# Autodesk Inventor assembly: HorquillaSuperior
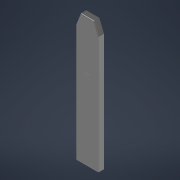
[picture p0: Inventor's stored thumbnail of the model, 180x180]
Saved by Autodesk Inventor 2022 (Build 260153000, 153)
## iProperties
Created: 2021-09-29
Part Number: HorquillaSuperior
Material: Generic
Document SubType Name: Assembly
Designer: Andres
Mass: 30510.4 g
Surface Area: 12356.1 cm^2
Volume: 3886.68 cm^3
Density: 7.85 g/cm^3
_SolveAssemblyDoc: Frame Generator Solve Assembly
_Version: 25.0.0
Author: Andres
## Documents named in this file (4)
- D:\Documentos\15.PUCP_2021-2\[PDM] Proyecto de Diseño Mecatrónico\ProyectoGIT\ProyectoRobotPallet\HorquillaSuperior\HorquillaSuperior.iam
- D:\Documentos\15.PUCP_2021-2\[PDM] Proyecto de Diseño Mecatrónico\ProyectoGIT\ProyectoRobotPallet\HorquillaSuperior\HorquillaSuperior.ipt
- D:\Documentos\15.PUCP_2021-2\[PDM] Proyecto de Diseño Mecatrónico\ProyectoGIT\ProyectoRobotPallet\HorquillaSuperior\HorquillaSuperior\Frame\Frame_HorqSup.iam
- D:\Documentos\15.PUCP_2021-2\[PDM] Proyecto de Diseño Mecatrónico\ProyectoGIT\ProyectoRobotPallet\HorquillaSuperior\PlanchaHorqSup.ipt
## Components (3 placed, 3 different names)
1. HorquillaSuperior:1
2. Frame_HorqSup:1 [sub-assembly] — Flush:1, Flush:2
3. PlanchaHorqSup:1 — Flush:1
## Relationships (2: Flush 2)
- Flush:1: Frame_HorqSup:1 ↔ PlanchaHorqSup:1
- Flush:2 (-120 mm): Frame_HorqSup:1
